# Autodesk Inventor assembly: ASY ДМФ лоток 050 илоотвод v2.0
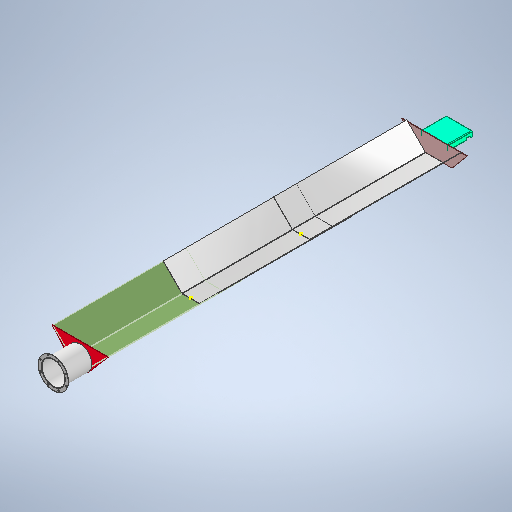
[picture p0: Inventor's stored thumbnail of the model, 512x512]
Saved by Autodesk Inventor 2026.2 (Build 302298000, 298)
## iProperties
Created: 2024-05-14
Part Number: ASY ДМФ лоток 050 илоотвод v2.0
Document SubType Name: Assembly
Designer: admin
Author: admin
## Documents named in this file (7)
- C:\Users\admin\Documents\Inventor\DMF-Disk-Micro-Filter\ASY ДМФ лоток 050 илоотвод v2.0.iam
- C:\Users\admin\Documents\Inventor\DMF-Disk-Micro-Filter\ДМФ 051 лоток илоотвод v2.0.ipt
- C:\Users\admin\Documents\Inventor\DMF-Disk-Micro-Filter\ДМФ 052 торец лотка кормовой v2.0.ipt
- C:\Users\admin\Documents\Inventor\DMF-Disk-Micro-Filter\ДМФ 053 швеллер лотка v2.0.ipt
- C:\Users\admin\Documents\Inventor\DMF-Disk-Micro-Filter\ДМФ 054 фланец лотка v2.0.ipt
- C:\Users\admin\Documents\Inventor\DMF-Disk-Micro-Filter\ДМФ 056 труба илоотвода v2.1.ipt
- C:\Users\admin\Documents\Inventor\DMF-Disk-Micro-Filter\Барабан v2.1\DMF 2.1 01 45 Gear ring 5_CPY1.ipt
## Components (8 placed, 7 different names)
1. ДМФ 051 лоток илоотвод v2.0.ipt:1 — Mate:2, Mate:3, Mate:4, Flush:3, Mate:5, Mate:6, Flush:4, Mate:7, Mate:12
2. ДМФ 052 торец лотка кормовой v2.0.ipt:1 — Rigid:2, Rigid:5
3. ДМФ 053 швеллер лотка v2.0.ipt:1 — Rigid:2
4. ДМФ 056 труба илоотвода v2.1:1 — Rigid:3, Rigid:4
5. ДМФ 054 фланец лотка v2.0.ipt:1 — Rigid:3, Mate:2, Mate:3, Mate:4, Flush:3, Mate:8
6. DMF 2.1 01 45 Gear ring 5_CPY1:1 — Rigid:4
7. ДМФ 051 лоток илоотвод v2.0:2 — Mate:5, Mate:6, Mate:9, Mate:10, Mate:11, Mate:12
8. ДМФ 051 лоток илоотвод v2.0:3 — Mate:9, Mate:10, Mate:11, Rigid:5
## Relationships (17: Mate 11, WeldJoint 4, Flush 2)
- Rigid:2 [WeldJoint]: ДМФ 052 торец лотка кормовой v2.0.ipt:1 ↔ ДМФ 053 швеллер лотка v2.0.ipt:1
- Rigid:3 [WeldJoint]: ДМФ 056 труба илоотвода v2.1:1 ↔ ДМФ 054 фланец лотка v2.0.ipt:1
- Mate:2: ДМФ 051 лоток илоотвод v2.0.ipt:1 ↔ ДМФ 054 фланец лотка v2.0.ipt:1
- Mate:3: ДМФ 051 лоток илоотвод v2.0.ipt:1 ↔ ДМФ 054 фланец лотка v2.0.ipt:1
- Mate:4: ДМФ 051 лоток илоотвод v2.0.ipt:1 ↔ ДМФ 054 фланец лотка v2.0.ipt:1
- Flush:3: ДМФ 051 лоток илоотвод v2.0.ipt:1 ↔ ДМФ 054 фланец лотка v2.0.ipt:1
- Mate:5: ДМФ 051 лоток илоотвод v2.0.ipt:1 ↔ ДМФ 051 лоток илоотвод v2.0:2
- Mate:6: ДМФ 051 лоток илоотвод v2.0.ipt:1 ↔ ДМФ 051 лоток илоотвод v2.0:2
- Flush:4: ДМФ 051 лоток илоотвод v2.0.ipt:1
- Mate:7: ДМФ 051 лоток илоотвод v2.0.ipt:1
- Mate:8: ДМФ 054 фланец лотка v2.0.ipt:1
- Rigid:4 [WeldJoint]: ДМФ 056 труба илоотвода v2.1:1 ↔ DMF 2.1 01 45 Gear ring 5_CPY1:1
- Mate:9: ДМФ 051 лоток илоотвод v2.0:2 ↔ ДМФ 051 лоток илоотвод v2.0:3
- Mate:10: ДМФ 051 лоток илоотвод v2.0:2 ↔ ДМФ 051 лоток илоотвод v2.0:3
- Mate:11: ДМФ 051 лоток илоотвод v2.0:2 ↔ ДМФ 051 лоток илоотвод v2.0:3
- Mate:12: ДМФ 051 лоток илоотвод v2.0.ipt:1 ↔ ДМФ 051 лоток илоотвод v2.0:2
- Rigid:5 [WeldJoint]: ДМФ 052 торец лотка кормовой v2.0.ipt:1 ↔ ДМФ 051 лоток илоотвод v2.0:3
